# Autodesk Inventor assembly: actuator
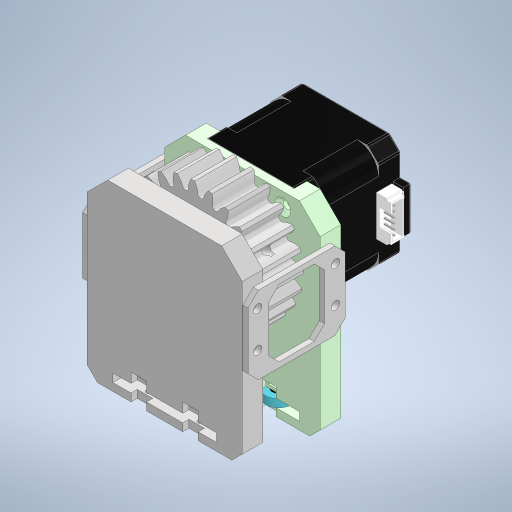
[picture p0: Inventor's stored thumbnail of the model, 512x512]
Saved by Autodesk Inventor 2023.1 (Build 271208000, 208)
## iProperties
Created: 2025-12-13
Part Number: actuator
Document SubType Name: Assembly
Designer: DELL
Author: DELL
## Documents named in this file (11)
- C:\Users\DELL\reposGitHub\VSOSH25-26\models\actuator\actuator.iam
- C:\Users\DELL\reposGitHub\VSOSH25-26\models\import\Schrittmotor-42SHDC3025-24B.ipt
- C:\Users\DELL\reposGitHub\VSOSH25-26\models\actuator\звезда_шестрерни.ipt
- C:\Users\DELL\reposGitHub\VSOSH25-26\models\actuator\муфта.ipt
- C:\Users\DELL\reposGitHub\VSOSH25-26\models\actuator\шестреня_12.12.ipt
- C:\Users\DELL\reposGitHub\VSOSH25-26\models\actuator\каретка.ipt
- C:\Users\DELL\reposGitHub\VSOSH25-26\models\actuator\колесико.ipt
- C:\Users\DELL\reposGitHub\VSOSH25-26\models\actuator\стена_простая.ipt
- C:\Users\DELL\reposGitHub\VSOSH25-26\models\import\222LX-Konstruktsionnyy-profil-20kh20L.ipt
- C:\Users\DELL\reposGitHub\VSOSH25-26\models\actuator\колесо.ipt
- C:\Users\DELL\reposGitHub\VSOSH25-26\models\actuator\каретка_м2_без_м.ipt
## Components (17 placed, 10 different names)
1. Schrittmotor-42SHDC3025-24B:1 — Заподлицо:1, Совмещение:1, Совмещение:2, Совмещение:4, Заподлицо:3
2. звезда_шестрерни:1 — Совмещение:5, Совмещение:6, Совмещение:7, Совмещение:8, Заподлицо:2
3. муфта:1 — Совмещение:4, Совмещение:5, Совмещение:6, Совмещение:9
4. шестреня_12.12:1 — Совмещение:7, Совмещение:8, Заподлицо:2
5. каретка:1 — Заподлицо:3, Совмещение:9, Совмещение:30, Совмещение:31, Совмещение:32, Совмещение:37, Совмещение:38, Заподлицо:4, Заподлицо:5, Совмещение:41, Совмещение:42, Совмещение:43, Совмещение:44
6. колесико:2 — Совмещение:40, Заподлицо:7, Совмещение:43
7. каретка:2 — Совмещение:34, Совмещение:36
8. колесико:3
9. колесико:4
10. стена_простая:1 — Совмещение:30, Совмещение:31, Совмещение:32, Совмещение:34, Совмещение:45, Совмещение:46
11. стена_простая:2 — Совмещение:36, Совмещение:37
12. 222LX-Konstruktsionnyy-profil-20kh20L:1 — Совмещение:38, Заподлицо:4, Заподлицо:5
13. колесо:1 — Совмещение:40, Заподлицо:7, Совмещение:44
14. колесо:2 — Совмещение:39, Заподлицо:6, Совмещение:42
15. колесико:5
16. колесико:6 — Совмещение:39, Заподлицо:6, Совмещение:41
17. каретка_м2_без_м:1 — Совмещение:45, Совмещение:46
## Relationships (30: Mate 23, Flush 7)
- Заподлицо:1 [Flush]: Schrittmotor-42SHDC3025-24B:1
- Совмещение:1 [Mate]: Schrittmotor-42SHDC3025-24B:1
- Совмещение:2 [Mate]: Schrittmotor-42SHDC3025-24B:1
- Совмещение:4 [Mate]: Schrittmotor-42SHDC3025-24B:1 ↔ муфта:1
- Совмещение:5 [Mate]: звезда_шестрерни:1 ↔ муфта:1
- Совмещение:6 [Mate]: звезда_шестрерни:1 ↔ муфта:1
- Совмещение:7 [Mate]: звезда_шестрерни:1 ↔ шестреня_12.12:1
- Совмещение:8 [Mate]: звезда_шестрерни:1 ↔ шестреня_12.12:1
- Заподлицо:2 [Flush]: звезда_шестрерни:1 ↔ шестреня_12.12:1
- Заподлицо:3 [Flush]: Schrittmotor-42SHDC3025-24B:1 ↔ каретка:1
- Совмещение:9 [Mate] (0.5 mm): муфта:1 ↔ каретка:1
- Совмещение:30 [Mate]: каретка:1 ↔ стена_простая:1
- Совмещение:31 [Mate]: каретка:1 ↔ стена_простая:1
- Совмещение:32 [Mate]: каретка:1 ↔ стена_простая:1
- Совмещение:34 [Mate]: каретка:2 ↔ стена_простая:1
- Совмещение:36 [Mate]: каретка:2 ↔ стена_простая:2
- Совмещение:37 [Mate]: каретка:1 ↔ стена_простая:2
- Совмещение:38 [Mate]: каретка:1 ↔ 222LX-Konstruktsionnyy-profil-20kh20L:1
- Заподлицо:4 [Flush]: каретка:1 ↔ 222LX-Konstruktsionnyy-profil-20kh20L:1
- Заподлицо:5 [Flush]: каретка:1 ↔ 222LX-Konstruktsionnyy-profil-20kh20L:1
- Совмещение:39 [Mate]: колесо:2 ↔ колесико:6
- Заподлицо:6 [Flush]: колесо:2 ↔ колесико:6
- Совмещение:40 [Mate]: колесико:2 ↔ колесо:1
- Заподлицо:7 [Flush]: колесико:2 ↔ колесо:1
- Совмещение:41 [Mate]: каретка:1 ↔ колесико:6
- Совмещение:42 [Mate]: каретка:1 ↔ колесо:2
- Совмещение:43 [Mate]: каретка:1 ↔ колесико:2
- Совмещение:44 [Mate]: каретка:1 ↔ колесо:1
- Совмещение:45 [Mate]: стена_простая:1 ↔ каретка_м2_без_м:1
- Совмещение:46 [Mate]: стена_простая:1 ↔ каретка_м2_без_м:1
